# Autodesk Inventor assembly: Bar Base Assembly
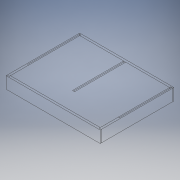
[picture p0: Inventor's stored thumbnail of the model, 180x180]
Saved by Autodesk Inventor 2016 (Build 200138000, 138)
## iProperties
Created: 2017-11-04
Part Number: Bar Base Assembly
Document SubType Name: Assembly
Designer: mathaetaes
Author: mathaetaes
## Documents named in this file (7)
- E:\Projects\3D Printer\printer projects\My Designs\Bar Cabinet 2.2.2018\Bar Base Assembly.iam
- E:\Projects\3D Printer\printer projects\My Designs\Bar Cabinet 2.2.2018\Bottom.ipt
- E:\Projects\3D Printer\printer projects\My Designs\Bar Cabinet 2.2.2018\Base Runner Side.ipt
- E:\Projects\3D Printer\printer projects\My Designs\Bar Cabinet 2.2.2018\Base Runner Front.ipt
- E:\Projects\3D Printer\printer projects\My Designs\Bar Cabinet 2.2.2018\Base Runner Side Right.ipt
- E:\Projects\3D Printer\printer projects\My Designs\Bar Cabinet 2.2.2018\Caster Block.ipt
- E:\Projects\3D Printer\printer projects\My Designs\Bar Cabinet 2.2.2018\Caster Placeholder.ipt
## Components (11 placed, 6 different names)
1. Bottom:1 — Mate:19, Mate:25, Mate:26, Mate:31, Mate:36, Mate:45, Mate:48, Mate:49, Mate:60, Flush:2, Flush:3
2. Base Runner Front:1 — Mate:25, Mate:26, Mate:37, Mate:46, Flush:2, Mate:61
3. Base Runner Side:1 — Mate:19, Mate:55, Mate:60, Flush:1
4. Base Runner Side Right:1 — Mate:31, Mate:53, Mate:54, Flush:1, Mate:61
5. Caster Block:2 — Mate:45, Mate:46, Mate:53, Mate:54, Mate:56, Mate:59
6. Caster Block:4 — Mate:36, Mate:37, Mate:55, Mate:57, Mate:58
7. Caster Placeholder:1 — Mate:59
8. Caster Placeholder:2 — Mate:56
9. Caster Placeholder:3 — Mate:57
10. Caster Placeholder:4 — Mate:58
11. Base Runner Front:2 — Mate:48, Mate:49, Flush:3
## Relationships (22: Mate 19, Flush 3)
- Mate:19: Bottom:1 ↔ Base Runner Side:1
- Mate:25: Bottom:1 ↔ Base Runner Front:1
- Mate:26: Bottom:1 ↔ Base Runner Front:1
- Mate:31: Bottom:1 ↔ Base Runner Side Right:1
- Mate:36: Bottom:1 ↔ Caster Block:4
- Mate:37: Base Runner Front:1 ↔ Caster Block:4
- Mate:45: Bottom:1 ↔ Caster Block:2
- Mate:46: Base Runner Front:1 ↔ Caster Block:2
- Mate:48: Bottom:1 ↔ Base Runner Front:2
- Mate:49: Bottom:1 ↔ Base Runner Front:2
- Mate:53: Base Runner Side Right:1 ↔ Caster Block:2
- Mate:54: Base Runner Side Right:1 ↔ Caster Block:2
- Mate:55: Base Runner Side:1 ↔ Caster Block:4
- Mate:56: Caster Block:2 ↔ Caster Placeholder:2
- Mate:57: Caster Block:4 ↔ Caster Placeholder:3
- Mate:58: Caster Block:4 ↔ Caster Placeholder:4
- Mate:59: Caster Block:2 ↔ Caster Placeholder:1
- Mate:60: Bottom:1 ↔ Base Runner Side:1
- Flush:1: Base Runner Side:1 ↔ Base Runner Side Right:1
- Flush:2: Bottom:1 ↔ Base Runner Front:1
- Mate:61: Base Runner Front:1 ↔ Base Runner Side Right:1
- Flush:3: Bottom:1 ↔ Base Runner Front:2
